# Autodesk Inventor assembly: High Strength 60-tooth Gear-Square Insert
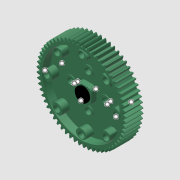
[picture p0: Inventor's stored thumbnail of the model, 180x180]
Saved by Autodesk Inventor 2021 (Build 250183000, 183)
## iProperties
Category: Motion
Company: Super Sonic Sparks, Team 24
Document SubType Name: Assembly
Designer: Jordan Kiesel
Vendor: VEX Robotics, Inc.
Description: Metal Square Hole Inserts prevent axles from "stripping".
Catalog Web Link: http://www.vexrobotics.com/products/accessories/motion/276-2250.html
Created: 2019-07-11
Author: Jordan Kiesel
Title: High Strength 60-tooth Gear-Square Insert
Comments: Build mechanisms capable of withstanding higher stresses than ever before. Lift heavier loads, and survive bigger impacts with high strength gears. ▷ High strength gears mate with all VEX spur gears. ▷ Double-thick face width provides added tooth strength. ▷ Metal Square Hole Inserts prevent axles from "stripping". ▷ Build gearboxes that resist high shock-loads. ▷ Bolt Gears together for added strength.
## Documents named in this file (3)
- E:\2020 BNS-VRC-SID-YY Library\Motion\Gears\High Strength 60-tooth Gear, Square Insert.iam
- E:\2020 BNS-VRC-SID-YY Library\Motion\Gears\Reference Parts\High Strength Gears\High Strength 60-Tooth Gear.ipt
- E:\2020 BNS-VRC-SID-YY Library\Motion\Reference Parts\High Strength Square Gear Insert.ipt
## Components (3 placed, 2 different names)
1. High Strength 60-Tooth Gear:1
2. High Strength Square Gear Insert:1
3. High Strength Square Gear Insert:2
## Relationships (6: Mate 6)
- [Mate]: High Strength 60-Tooth Gear:1 ↔ High Strength Square Gear Insert:1
- [Mate] (0.0254 mm): High Strength 60-Tooth Gear:1 ↔ High Strength Square Gear Insert:1
- [Mate] (0.0254 mm): High Strength 60-Tooth Gear:1 ↔ High Strength Square Gear Insert:1
- [Mate]: High Strength 60-Tooth Gear:1 ↔ High Strength Square Gear Insert:2
- [Mate] (0.0254 mm): High Strength 60-Tooth Gear:1 ↔ High Strength Square Gear Insert:2
- [Mate] (0.0254 mm): High Strength 60-Tooth Gear:1 ↔ High Strength Square Gear Insert:2
